# Autodesk Inventor assembly: ParkingTapeRedFull
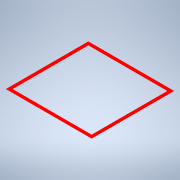
[picture p0: Inventor's stored thumbnail of the model, 180x180]
Saved by Autodesk Inventor 2021 (Build 250183000, 183)
## iProperties
Created: 2021-03-04
Part Number: ParkingTapeRedFull
Document SubType Name: Assembly
Designer: CMurray
Author: CMurray
## Documents named in this file (2)
- F:\PHRC CADD 2021\2021 Game Design Challenge\Full Field\Parts\Tape\ParkingTapeRedFull.iam
- F:\PHRC CADD 2021\2021 Game Design Challenge\Full Field\Parts\Tape\BlueParkingTape.ipt
## Components (4 placed, 1 different names)
1. BlueParkingTape:1 — Flush:1, Mate:1, Flush:2, Mate:3
2. BlueParkingTape:2 — Flush:1, Mate:1, Flush:2, Mate:2, Flush:3, Flush:4
3. BlueParkingTape:3 — Mate:2, Flush:3, Flush:4, Flush:5, Flush:6
4. BlueParkingTape:4 — Flush:5, Flush:6, Mate:3
## Relationships (9: Flush 6, Mate 3)
- Flush:1: BlueParkingTape:1 ↔ BlueParkingTape:2
- Mate:1: BlueParkingTape:1 ↔ BlueParkingTape:2
- Flush:2: BlueParkingTape:1 ↔ BlueParkingTape:2
- Mate:2: BlueParkingTape:2 ↔ BlueParkingTape:3
- Flush:3: BlueParkingTape:2 ↔ BlueParkingTape:3
- Flush:4: BlueParkingTape:2 ↔ BlueParkingTape:3
- Flush:5: BlueParkingTape:3 ↔ BlueParkingTape:4
- Flush:6: BlueParkingTape:3 ↔ BlueParkingTape:4
- Mate:3: BlueParkingTape:1 ↔ BlueParkingTape:4
